# Autodesk Inventor assembly: BOLTWASHER3X16
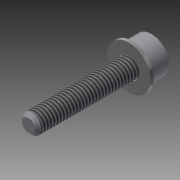
[picture p0: Inventor's stored thumbnail of the model, 180x180]
Saved by Autodesk Inventor 2015 SP1 (Build 190203100, 203)
## iProperties
Category: Hardware
Created: 2015-01-16
Part Number: BOLTWASHER3X16
Document SubType Name: Assembly
Designer: Jack
Mass: 0.282444 g
Surface Area: 3.34363 cm^2
Volume: 0.186107 cm^3
Density: 1.51765 g/cm^3
Vendor: Misumi
Author: Jack
Title: Bolt + Washer 3x16
## Documents named in this file (3)
- C:\Users\Jack\ownCloud\Projects\CrossBot\InventorModel\Hardware\BoltWashers\BoltWasher3\BoltWasher3x16.iam
- C:\Users\Jack\ownCloud\Projects\CrossBot\InventorModel\Hardware\Wahsers\M3Washer.ipt
- C:\Users\Jack\ownCloud\Projects\CrossBot\InventorModel\Hardware\Bolts\SHCS\SHCS3\SHCS3x16.ipt
## Components (2 placed, 2 different names)
1. M3Washer:1 — Mate:1, Mate:2
2. SHCS3x16:1 — Mate:1, Mate:2
## Relationships (2: Mate 2)
- Mate:1: M3Washer:1 ↔ SHCS3x16:1
- Mate:2: M3Washer:1 ↔ SHCS3x16:1
